# Autodesk Inventor assembly: Pusher
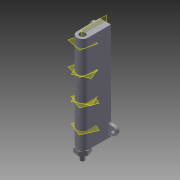
[picture p0: Inventor's stored thumbnail of the model, 180x180]
Saved by Autodesk Inventor 2011 (Build 150239000, 239)
## iProperties
Created: 2011-04-01
Part Number: Pusher
Document SubType Name: Assembly
Designer: Rob
Author: Rob
## Documents named in this file (6)
- C:\Users\Rob\Dropbox\RockSAT-X 2011 RexSAT\capsule-launcher.design\Launcher\Pusher.iam
- C:\Users\Rob\Dropbox\RockSAT-X 2011 RexSAT\capsule-launcher.design\Launcher\Pusher.Holder.ipt
- C:\Users\Rob\Dropbox\RockSAT-X 2011 RexSAT\capsule-launcher.design\Launcher\Pusher.Pushrod.ipt
- C:\Users\Rob\Dropbox\RockSAT-X 2011 RexSAT\capsule-launcher.design\Launcher\Pusher.springplate.ipt
- C:\Users\Rob\Dropbox\RockSAT-X 2011 RexSAT\capsule-launcher.design\Launcher\Pusher.Bolt.ipt
- C:\Users\Rob\Dropbox\RockSAT-X 2011 RexSAT\capsule-launcher.design\Launcher\Pusher.Spring(long).ipt
## Components (9 placed, 5 different names)
1. Pusher.Holder:1 — Mate:1, Mate:2, Mate:4, Mate:12, Mate:13, Mate:14, Mate:17
2. Pusher.Pushrod:1 — Mate:1, Mate:3, Flush:4
3. Pusher.springplate:1 — Mate:2, Mate:15, Flush:2
4. Pusher.Bolt:1 — Mate:3, Mate:4, Flush:4
5. Pusher.springplate:2 — Mate:12, Mate:16, Flush:3
6. Pusher.Spring(long):1 — Mate:13, Mate:15
7. Pusher.Spring(long):2 — Mate:14, Flush:2, Mate:16
8. Pusher.Spring(long):3 — Mate:17, Flush:3, Mate:18, Mate:19
9. Pusher.springplate:3 — Mate:18, Mate:19
## Relationships (15: Mate 12, Flush 3)
- Mate:1: Pusher.Holder:1 ↔ Pusher.Pushrod:1
- Mate:2: Pusher.Holder:1 ↔ Pusher.springplate:1
- Mate:3: Pusher.Pushrod:1 ↔ Pusher.Bolt:1
- Mate:4: Pusher.Holder:1 ↔ Pusher.Bolt:1
- Mate:12: Pusher.Holder:1 ↔ Pusher.springplate:2
- Mate:13: Pusher.Holder:1 ↔ Pusher.Spring(long):1
- Mate:14: Pusher.Holder:1 ↔ Pusher.Spring(long):2
- Mate:15: Pusher.springplate:1 ↔ Pusher.Spring(long):1
- Flush:2: Pusher.springplate:1 ↔ Pusher.Spring(long):2
- Mate:16: Pusher.springplate:2 ↔ Pusher.Spring(long):2
- Mate:17: Pusher.Holder:1 ↔ Pusher.Spring(long):3
- Flush:3: Pusher.springplate:2 ↔ Pusher.Spring(long):3
- Mate:18: Pusher.Spring(long):3 ↔ Pusher.springplate:3
- Mate:19: Pusher.Spring(long):3 ↔ Pusher.springplate:3
- Flush:4 (-10 mm): Pusher.Pushrod:1 ↔ Pusher.Bolt:1
